# Autodesk Inventor assembly: wall_glides
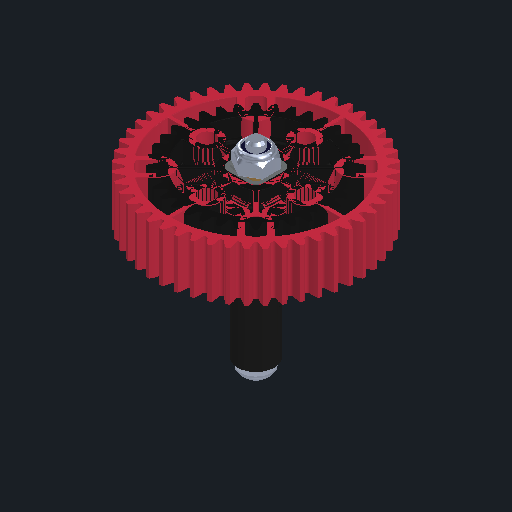
[picture p0: Inventor's stored thumbnail of the model, 512x512]
Saved by Autodesk Inventor 2025 (Build 290162000, 162)
## iProperties
Created: 2024-08-21
Part Number: wall_glides
Document SubType Name: Assembly
Designer: averey
Author: averey
## Documents named in this file (11)
- D:\vex_robotics_high_stakes\hardware\cad\bots\ENIGMA\chassis\drivetrain\drivebay\wall_glides.iam
- D:\vex_robotics_high_stakes\hardware\cad\VEX-CAD-Inventor\Motion\Spacers\Spacer Nylon .375 OD\NSpacer .375 OD x .500.ipt
- C:\Users\avere\vex_robotics_high_stakes\hardware\cad\VEX-CAD-Inventor\Motion\Spacers\Spacer Nylon .375 OD.ipt
- D:\vex_robotics_high_stakes\hardware\cad\VEX-CAD-Inventor\Motion\Gears\HS Gear\HS 36T Gear, Circle.iam
- C:\Users\avere\vex_robotics_high_stakes\hardware\cad\VEX-CAD-Inventor\Motion\Gears\HS Gear.iam
- D:\vex_robotics_high_stakes\hardware\cad\VEX-CAD-Inventor\Structure\Hardware\Nut Thin Nylock.ipt
- D:\vex_robotics_high_stakes\hardware\cad\VEX-CAD-Inventor\Structure\Hardware\Nut Nylon\Nut Nylon - White.ipt
- C:\Users\avere\vex_robotics_high_stakes\hardware\cad\VEX-CAD-Inventor\Structure\Hardware\Nut Nylon.ipt
- D:\vex_robotics_high_stakes\hardware\cad\VEX-CAD-Inventor\Structure\Hardware\Screw Shoulder Robosource\SScrew Shoulder Smooth 2.000 x .04.ipt
- C:\Users\avere\vex_robotics_high_stakes\hardware\cad\VEX-CAD-Inventor\Structure\Hardware\Screw Shoulder Robosource.ipt
- D:\vex_robotics_high_stakes\hardware\cad\VEX-CAD-Inventor\Motion\Gears\HS Gear\HS 48T Gear, Circle.iam
## Components (7 placed, 6 different names)
1. NSpacer .375 OD x .500:1 — Insert:4
2. NSpacer .375 OD x .500:2 — Insert:5
3. HS 36T Gear, Circle:1 [sub-assembly] — Insert:6
4. Nut Thin Nylock:1
5. Nut Nylon - White:1 — Insert:5, Mate:1
6. SScrew Shoulder Smooth 2.000 x .04:1 — Insert:4
7. HS 48T Gear, Circle:2 [sub-assembly] — Insert:6
## Relationships (7: Insert 6, Mate 1)
- [Insert]: NSpacer .375 OD x .500:1 ↔ NSpacer .375 OD x .500:2
- [Insert]: HS 36T Gear, Circle:1 ↔ Nut Thin Nylock:1
- [Insert]: HS 36T Gear, Circle:1 ↔ Nut Nylon - White:1
- Insert:4 (1.5875 mm): NSpacer .375 OD x .500:1 ↔ SScrew Shoulder Smooth 2.000 x .04:1
- Insert:5 (1.5875 mm): NSpacer .375 OD x .500:2 ↔ Nut Nylon - White:1
- Mate:1: Nut Nylon - White:1
- Insert:6: HS 36T Gear, Circle:1 ↔ HS 48T Gear, Circle:2
